# Autodesk Inventor assembly: Blade
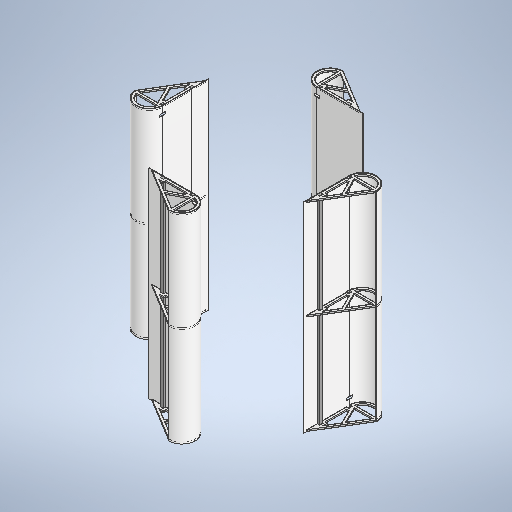
[picture p0: Inventor's stored thumbnail of the model, 512x512]
Saved by Autodesk Inventor 2025.1 (Build 291241000, 241)
## iProperties
Created: 2025-01-28
Part Number: Blade
Document SubType Name: Assembly
Designer: Dimas Arif
Author: Dimas Arif
## Documents named in this file (4)
- C:\Users\Dimas Arif\Documents\Inventor\Project-81\Blade.iam
- C:\Users\Dimas Arif\Documents\Inventor\Project-81\Balde.ipt
- C:\Users\Dimas Arif\Documents\Inventor\Project-81\F1.ipt
- C:\Users\Dimas Arif\Documents\Inventor\Project-81\P1.ipt
## Components (20 placed, 3 different names)
1. Balde:1 — Flush:1, Flush:3, Flush:4
2. F1:1 — Mate:1, Mate:2, Flush:2
3. Balde:2
4. F1:2
5. Balde:3
6. F1:3
7. Balde:4
8. F1:4
9. P1:1 — Flush:1, Mate:1, Mate:2, Flush:2
10. P1:2 — Symmetry:1
11. P1:3
12. P1:4
13. P1:5
14. P1:6
15. P1:7
16. P1:8 — Symmetry:1
17. P1:9
18. P1:10
19. P1:11
20. P1:12
## Component patterns: (4 elements, first: Balde:1 + F1:1), (3 elements, first: P1:1), Component Pattern 1:2 (3 elements), Component Pattern 1:3 (3 elements), Component Pattern 1:4 (3 elements)
## Relationships (9: Flush 4, Mate 4, Symmetry 1)
- Flush:1: Balde:1 ↔ P1:1
- Mate:1: F1:1 ↔ P1:1
- Mate:2: F1:1 ↔ P1:1
- Flush:2: F1:1 ↔ P1:1
- Flush:3 (500 mm): Balde:1
- Flush:4 (-194 mm): Balde:1
- Mate:3
- Mate:4
- Symmetry:1: P1:2 ↔ P1:8
